# Autodesk Inventor assembly: capoAsm
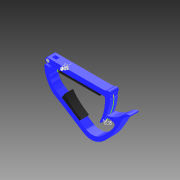
[picture p0: Inventor's stored thumbnail of the model, 180x180]
Saved by Autodesk Inventor 2012 (Build 160160000, 160)
## iProperties
Created: 2013-08-01
Part Number: capoAsm
Document SubType Name: Assembly
Designer: Dantro
Author: Dantro
## Documents named in this file (6)
- D:\testFiles\Inventor\Capo\capoAsm.iam
- D:\testFiles\Inventor\Capo\capo1.ipt
- D:\testFiles\Inventor\Capo\capo2.ipt
- D:\testFiles\Inventor\Capo\fix.ipt
- D:\testFiles\Inventor\Capo\ruber1.ipt
- D:\testFiles\Inventor\Capo\ruber2.ipt
## Components (5 placed, 5 different names)
1. capo1:1 — Mate:1, Flush:1, Mate:2, Mate:3, Mate:5, Flush:2
2. capo2:1 — Mate:1, Flush:1, Mate:4, Flush:3
3. fix:1 — Mate:2, Mate:3
4. ruber1:1 — Mate:4, Flush:3
5. ruber2:1 — Mate:5, Flush:2
## Relationships (8: Mate 5, Flush 3)
- Mate:1: capo1:1 ↔ capo2:1
- Flush:1: capo1:1 ↔ capo2:1
- Mate:2: capo1:1 ↔ fix:1
- Mate:3: capo1:1 ↔ fix:1
- Mate:4: capo2:1 ↔ ruber1:1
- Mate:5: capo1:1 ↔ ruber2:1
- Flush:2 (0.5 mm): capo1:1 ↔ ruber2:1
- Flush:3 (0.25 mm): capo2:1 ↔ ruber1:1
